# Autodesk Inventor assembly: assamblage_demo
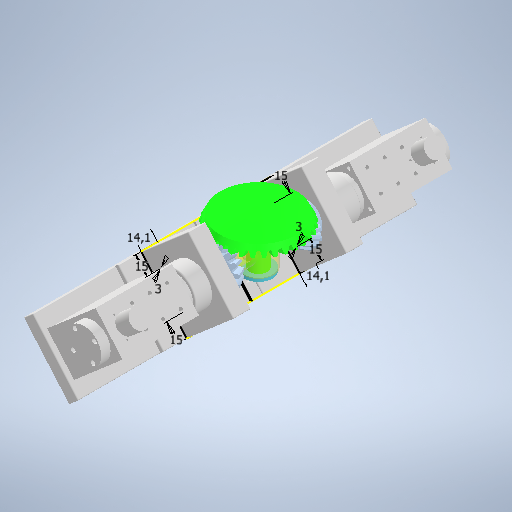
[picture p0: Inventor's stored thumbnail of the model, 512x512]
Saved by Autodesk Inventor 2025.1 (Build 291241000, 241)
## iProperties
Created: 2025-07-18
Part Number: assamblage_demo
Document SubType Name: Assembly
Designer: chapuzet
Author: chapuzet
## Documents named in this file (12)
- C:\Users\chapuzet\Documents\stage_ensta_rai\mecanique_robot_raie\base_meca\systeme_reference\demo_filament+usinage\assamblage_demo.iam
- C:\Users\chapuzet\Documents\stage_ensta_rai\mecanique_robot_raie\base_meca\systeme_reference\demo_filament+usinage\axe_central_demo.ipt
- C:\Users\chapuzet\Documents\stage_ensta_rai\mecanique_robot_raie\base_meca\systeme_reference\demo_filament+usinage\Cross_demo_mod.ipt
- C:\Users\chapuzet\Documents\stage_ensta_rai\mecanique_robot_raie\base_meca\systeme_reference\demo_filament+usinage\demi_socle_demo.ipt
- C:\Users\chapuzet\Documents\stage_ensta_rai\mecanique_robot_raie\base_meca\systeme_reference\demo_filament+usinage\engrenage_secondaire_demo.ipt
- C:\Users\chapuzet\Documents\stage_ensta_rai\mecanique_robot_raie\base_meca\systeme_reference\demo_filament+usinage\extremite_axe_central_demo.ipt
- C:\Users\chapuzet\Documents\stage_ensta_rai\mecanique_robot_raie\base_meca\systeme_reference\demo_filament+usinage\fixation_harbre_moteur_demo.ipt
- C:\Users\chapuzet\Documents\stage_ensta_rai\mecanique_robot_raie\base_meca\systeme_reference\demo_filament+usinage\jonction_demi_socle_demo.ipt
- C:\Users\chapuzet\Documents\stage_ensta_rai\mecanique_robot_raie\base_meca\systeme_reference\demo_filament+usinage\plaque_soutient_demo.ipt
- C:\Users\chapuzet\Documents\stage_ensta_rai\mecanique_robot_raie\base_meca\Servo_moteur_rovmaker.ipt
- C:\Users\chapuzet\Documents\stage_ensta_rai\mecanique_robot_raie\base_meca\systeme_reference\demo_filament+usinage\screw_gb_t_70_1_m4x12.ipt
- C:\Users\chapuzet\Documents\stage_ensta_rai\mecanique_robot_raie\base_meca\systeme_reference\demo_filament+usinage\screw_gb_t_2674_m3x16_conique.ipt
## Components (34 placed, 11 different names)
1. axe_central_demo:1 — Cylindrique:3, Placage:30, Placage:32, Placage:33
2. Cross_demo_mod:1 — Cylindrique:1, Cylindrique:2, Placage:29, Cylindrique:3, Placage:30, Placage:31
3. demi_socle_demo:1 — Placage:3, Placage:5, Placage:6, Placage:7, Placage:8, Placage:9, Placage:19, Placage:20, Placage:21, Placage:40, Placage:41, Placage:42, Placage:43, Placage:44, Placage:45, Placage:52, Placage:53, Placage:54, Placage:55, Placage:56, Placage:57
4. engrenage_secondaire_demo:1 — Placage:27, Placage:28, Cylindrique:1
5. extremite_axe_central_demo:1 — Placage:31, Placage:32, Placage:33
6. fixation_harbre_moteur_demo:1 — Placage:13, Placage:14, Placage:15, Placage:66, Placage:67, Placage:68, Placage:69, Placage:70, Placage:71, Placage:72, Placage:73
7. jonction_demi_socle_demo:1 — Placage:1, Placage:2, Placage:3, Placage:4, Placage:5, Placage:6
8. plaque_soutient_demo:1 — Placage:10, Placage:11, Placage:12, Placage:27, Placage:28
9. demi_socle_demo:2 — Placage:1, Placage:2, Placage:4, Placage:10, Placage:11, Placage:12, Placage:22, Placage:23, Placage:24, Placage:34, Placage:35, Placage:36, Placage:37, Placage:38, Placage:39, Placage:46, Placage:47, Placage:48, Placage:49, Placage:50, Placage:51
10. engrenage_secondaire_demo:2 — Placage:25, Placage:26, Cylindrique:2, Placage:29
11. fixation_harbre_moteur_demo:2 — Placage:16, Placage:17, Placage:18, Placage:58, Placage:59, Placage:60, Placage:61, Placage:62, Placage:63, Placage:64, Placage:65
12. plaque_soutient_demo:2 — Placage:7, Placage:8, Placage:9, Placage:25, Placage:26
13. Servo_moteur_rovmaker:1 — Placage:16, Placage:17, Placage:18, Placage:19, Placage:20, Placage:21
14. Servo_moteur_rovmaker:2 — Placage:13, Placage:14, Placage:15, Placage:22, Placage:23, Placage:24
15. screw_gb_t_2674_m3x16_conique:2 — Placage:34, Placage:46
16. screw_gb_t_2674_m3x16_conique:3 — Placage:35, Placage:51
17. screw_gb_t_2674_m3x16_conique:4 — Placage:36, Placage:47
18. screw_gb_t_2674_m3x16_conique:5 — Placage:37, Placage:50
19. screw_gb_t_2674_m3x16_conique:6 — Placage:38, Placage:49
20. screw_gb_t_2674_m3x16_conique:7 — Placage:39, Placage:48
21. screw_gb_t_2674_m3x16_conique:8 — Placage:40, Placage:57
22. screw_gb_t_2674_m3x16_conique:9 — Placage:41, Placage:56
23. screw_gb_t_2674_m3x16_conique:10 — Placage:42, Placage:54
24. screw_gb_t_2674_m3x16_conique:11 — Placage:43, Placage:53
25. screw_gb_t_2674_m3x16_conique:12 — Placage:44, Placage:55
26. screw_gb_t_2674_m3x16_conique:13 — Placage:45, Placage:52
27. screw_gb_t_70_1_m4x12:1 — Placage:61, Placage:64
28. screw_gb_t_70_1_m4x12:2 — Placage:60, Placage:63
29. screw_gb_t_70_1_m4x12:3 — Placage:59, Placage:65
30. screw_gb_t_70_1_m4x12:4 — Placage:58, Placage:62
31. screw_gb_t_70_1_m4x12:5 — Placage:66, Placage:71
32. screw_gb_t_70_1_m4x12:6 — Placage:67, Placage:70
33. screw_gb_t_70_1_m4x12:7 — Placage:68, Placage:73
34. screw_gb_t_70_1_m4x12:8 — Placage:69, Placage:72
## Relationships (76: Mate 73, CylindricalJoint 3)
- Placage:1 [Mate]: jonction_demi_socle_demo:1 ↔ demi_socle_demo:2
- Placage:2 [Mate]: jonction_demi_socle_demo:1 ↔ demi_socle_demo:2
- Placage:3 [Mate]: demi_socle_demo:1 ↔ jonction_demi_socle_demo:1
- Placage:4 [Mate]: jonction_demi_socle_demo:1 ↔ demi_socle_demo:2
- Placage:5 [Mate]: demi_socle_demo:1 ↔ jonction_demi_socle_demo:1
- Placage:6 [Mate]: demi_socle_demo:1 ↔ jonction_demi_socle_demo:1
- Placage:7 [Mate]: demi_socle_demo:1 ↔ plaque_soutient_demo:2
- Placage:8 [Mate]: demi_socle_demo:1 ↔ plaque_soutient_demo:2
- Placage:9 [Mate]: demi_socle_demo:1 ↔ plaque_soutient_demo:2
- Placage:10 [Mate]: plaque_soutient_demo:1 ↔ demi_socle_demo:2
- Placage:11 [Mate]: plaque_soutient_demo:1 ↔ demi_socle_demo:2
- Placage:12 [Mate]: plaque_soutient_demo:1 ↔ demi_socle_demo:2
- Placage:13 [Mate]: fixation_harbre_moteur_demo:1 ↔ Servo_moteur_rovmaker:2
- Placage:14 [Mate]: fixation_harbre_moteur_demo:1 ↔ Servo_moteur_rovmaker:2
- Placage:15 [Mate]: fixation_harbre_moteur_demo:1 ↔ Servo_moteur_rovmaker:2
- Placage:16 [Mate]: fixation_harbre_moteur_demo:2 ↔ Servo_moteur_rovmaker:1
- Placage:17 [Mate]: fixation_harbre_moteur_demo:2 ↔ Servo_moteur_rovmaker:1
- Placage:18 [Mate]: fixation_harbre_moteur_demo:2 ↔ Servo_moteur_rovmaker:1
- Placage:19 [Mate]: demi_socle_demo:1 ↔ Servo_moteur_rovmaker:1
- Placage:20 [Mate]: demi_socle_demo:1 ↔ Servo_moteur_rovmaker:1
- Placage:21 [Mate]: demi_socle_demo:1 ↔ Servo_moteur_rovmaker:1
- Placage:22 [Mate]: demi_socle_demo:2 ↔ Servo_moteur_rovmaker:2
- Placage:23 [Mate]: demi_socle_demo:2 ↔ Servo_moteur_rovmaker:2
- Placage:24 [Mate]: demi_socle_demo:2 ↔ Servo_moteur_rovmaker:2
- Placage:25 [Mate]: engrenage_secondaire_demo:2 ↔ plaque_soutient_demo:2
- Placage:26 [Mate] (-1 mm): engrenage_secondaire_demo:2 ↔ plaque_soutient_demo:2
- Placage:27 [Mate]: engrenage_secondaire_demo:1 ↔ plaque_soutient_demo:1
- Placage:28 [Mate] (-1 mm): engrenage_secondaire_demo:1 ↔ plaque_soutient_demo:1
- Cylindrique:1: Cross_demo_mod:1 ↔ engrenage_secondaire_demo:1
- Cylindrique:2: Cross_demo_mod:1 ↔ engrenage_secondaire_demo:2
- Placage:29 [Mate] (0.5 mm): Cross_demo_mod:1 ↔ engrenage_secondaire_demo:2
- Cylindrique:3: axe_central_demo:1 ↔ Cross_demo_mod:1
- Placage:30 [Mate]: axe_central_demo:1 ↔ Cross_demo_mod:1
- Placage:31 [Mate]: Cross_demo_mod:1 ↔ extremite_axe_central_demo:1
- Placage:32 [Mate]: axe_central_demo:1 ↔ extremite_axe_central_demo:1
- Placage:33 [Mate]: axe_central_demo:1 ↔ extremite_axe_central_demo:1
- Placage:34 [Mate]: demi_socle_demo:2 ↔ screw_gb_t_2674_m3x16_conique:2
- Placage:35 [Mate]: demi_socle_demo:2 ↔ screw_gb_t_2674_m3x16_conique:3
- Placage:36 [Mate]: demi_socle_demo:2 ↔ screw_gb_t_2674_m3x16_conique:4
- Placage:37 [Mate]: demi_socle_demo:2 ↔ screw_gb_t_2674_m3x16_conique:5
- Placage:38 [Mate]: demi_socle_demo:2 ↔ screw_gb_t_2674_m3x16_conique:6
- Placage:39 [Mate]: demi_socle_demo:2 ↔ screw_gb_t_2674_m3x16_conique:7
- Placage:40 [Mate]: demi_socle_demo:1 ↔ screw_gb_t_2674_m3x16_conique:8
- Placage:41 [Mate]: demi_socle_demo:1 ↔ screw_gb_t_2674_m3x16_conique:9
- Placage:42 [Mate]: demi_socle_demo:1 ↔ screw_gb_t_2674_m3x16_conique:10
- Placage:43 [Mate]: demi_socle_demo:1 ↔ screw_gb_t_2674_m3x16_conique:11
- Placage:44 [Mate]: demi_socle_demo:1 ↔ screw_gb_t_2674_m3x16_conique:12
- Placage:45 [Mate]: demi_socle_demo:1 ↔ screw_gb_t_2674_m3x16_conique:13
- Placage:46 [Mate]: demi_socle_demo:2 ↔ screw_gb_t_2674_m3x16_conique:2
- Placage:47 [Mate]: demi_socle_demo:2 ↔ screw_gb_t_2674_m3x16_conique:4
- Placage:48 [Mate]: demi_socle_demo:2 ↔ screw_gb_t_2674_m3x16_conique:7
- Placage:49 [Mate]: demi_socle_demo:2 ↔ screw_gb_t_2674_m3x16_conique:6
- Placage:50 [Mate]: demi_socle_demo:2 ↔ screw_gb_t_2674_m3x16_conique:5
- Placage:51 [Mate]: demi_socle_demo:2 ↔ screw_gb_t_2674_m3x16_conique:3
- Placage:52 [Mate]: demi_socle_demo:1 ↔ screw_gb_t_2674_m3x16_conique:13
- Placage:53 [Mate]: demi_socle_demo:1 ↔ screw_gb_t_2674_m3x16_conique:11
- Placage:54 [Mate]: demi_socle_demo:1 ↔ screw_gb_t_2674_m3x16_conique:10
- Placage:55 [Mate]: demi_socle_demo:1 ↔ screw_gb_t_2674_m3x16_conique:12
- Placage:56 [Mate]: demi_socle_demo:1 ↔ screw_gb_t_2674_m3x16_conique:9
- Placage:57 [Mate]: demi_socle_demo:1 ↔ screw_gb_t_2674_m3x16_conique:8
- Placage:58 [Mate]: fixation_harbre_moteur_demo:2 ↔ screw_gb_t_70_1_m4x12:4
- Placage:59 [Mate]: fixation_harbre_moteur_demo:2 ↔ screw_gb_t_70_1_m4x12:3
- Placage:60 [Mate]: fixation_harbre_moteur_demo:2 ↔ screw_gb_t_70_1_m4x12:2
- Placage:61 [Mate]: fixation_harbre_moteur_demo:2 ↔ screw_gb_t_70_1_m4x12:1
- Placage:62 [Mate]: fixation_harbre_moteur_demo:2 ↔ screw_gb_t_70_1_m4x12:4
- Placage:63 [Mate]: fixation_harbre_moteur_demo:2 ↔ screw_gb_t_70_1_m4x12:2
- Placage:64 [Mate]: fixation_harbre_moteur_demo:2 ↔ screw_gb_t_70_1_m4x12:1
- Placage:65 [Mate]: fixation_harbre_moteur_demo:2 ↔ screw_gb_t_70_1_m4x12:3
- Placage:66 [Mate]: fixation_harbre_moteur_demo:1 ↔ screw_gb_t_70_1_m4x12:5
- Placage:67 [Mate]: fixation_harbre_moteur_demo:1 ↔ screw_gb_t_70_1_m4x12:6
- Placage:68 [Mate]: fixation_harbre_moteur_demo:1 ↔ screw_gb_t_70_1_m4x12:7
- Placage:69 [Mate]: fixation_harbre_moteur_demo:1 ↔ screw_gb_t_70_1_m4x12:8
- Placage:70 [Mate]: fixation_harbre_moteur_demo:1 ↔ screw_gb_t_70_1_m4x12:6
- Placage:71 [Mate]: fixation_harbre_moteur_demo:1 ↔ screw_gb_t_70_1_m4x12:5
- Placage:72 [Mate]: fixation_harbre_moteur_demo:1 ↔ screw_gb_t_70_1_m4x12:8
- Placage:73 [Mate]: fixation_harbre_moteur_demo:1 ↔ screw_gb_t_70_1_m4x12:7
